# Autodesk Inventor assembly: Body Xu4
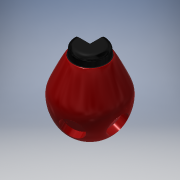
[picture p0: Inventor's stored thumbnail of the model, 180x180]
Saved by Autodesk Inventor 2018 (Build 220112000, 112)
## iProperties
Created: 2017-08-21
Part Number: Body Xu4
Material: Generisch
Document SubType Name: Assembly
Designer: JochenAlt
Author: JochenAlt
## Documents named in this file (8)
- D:\Projects\Manfred\design\cad\Inventor\Body Xu4.iam
- D:\Projects\Manfred\design\cad\Inventor\Body.ipt
- D:\Projects\Manfred\design\cad\Inventor\ODroid Xu4 Holder.ipt
- D:\Projects\Manfred\design\cad\Inventor\Odroid-XU4.ipt
- D:\Projects\Manfred\design\cad\Inventor\Lidar-Holder-xu4.ipt
- D:\Projects\Manfred\design\cad\Inventor\BNO055.ipt
- D:\Projects\Manfred\design\cad\Inventor\RPLidar A2.ipt
- D:\Projects\Manfred\design\cad\Inventor\PCB Slamtec RPLidar A2.ipt
## Components (7 placed, 7 different names)
1. Body:1 — Passend:1, Winkel:1, Passend:2
2. ODroid Xu4 Holder:1 — Passend:1, Winkel:1, Passend:2, Passend:3, Passend:4, Passend:5, Winkel:2, Passend:6
3. Odroid-XU4:1 — Passend:3, Passend:4
4. Lidar-Holder-xu4:1 — Passend:5, Winkel:2, Passend:6, Passend:8, Passend:9, Passend:10, Passend:11, Passend:12, Passend:13
5. BNO055:1 — Passend:8
6. RPLidar A2:1 — Passend:9, Passend:10, Passend:11
7. PCB Slamtec RPLidar A2:1 — Passend:12, Passend:13
## Relationships (14: Mate 12, Angle 2)
- Passend:1 [Mate]: Body:1 ↔ ODroid Xu4 Holder:1
- Winkel:1 [Angle] (180 deg): Body:1 ↔ ODroid Xu4 Holder:1
- Passend:2 [Mate] (0.1 mm): Body:1 ↔ ODroid Xu4 Holder:1
- Passend:3 [Mate]: ODroid Xu4 Holder:1 ↔ Odroid-XU4:1
- Passend:4 [Mate]: ODroid Xu4 Holder:1 ↔ Odroid-XU4:1
- Passend:5 [Mate]: ODroid Xu4 Holder:1 ↔ Lidar-Holder-xu4:1
- Winkel:2 [Angle] (180 deg): ODroid Xu4 Holder:1 ↔ Lidar-Holder-xu4:1
- Passend:6 [Mate] (0.1 mm): ODroid Xu4 Holder:1 ↔ Lidar-Holder-xu4:1
- Passend:8 [Mate]: Lidar-Holder-xu4:1 ↔ BNO055:1
- Passend:9 [Mate]: Lidar-Holder-xu4:1 ↔ RPLidar A2:1
- Passend:10 [Mate]: Lidar-Holder-xu4:1 ↔ RPLidar A2:1
- Passend:11 [Mate]: Lidar-Holder-xu4:1 ↔ RPLidar A2:1
- Passend:12 [Mate]: Lidar-Holder-xu4:1 ↔ PCB Slamtec RPLidar A2:1
- Passend:13 [Mate]: Lidar-Holder-xu4:1 ↔ PCB Slamtec RPLidar A2:1
